# Autodesk Inventor assembly: Top PVC Roller
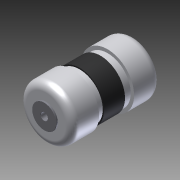
[picture p0: Inventor's stored thumbnail of the model, 180x180]
Saved by Autodesk Inventor 2014 SP1 (Build 180222100, 222)
## iProperties
Created: 2012-03-30
Part Number: Top PVC Roller
Document SubType Name: Assembly
Designer: Moses
Author: Moses
## Documents named in this file (5)
- C:\Users\Moses\Documents\Inventor\Rebuild\Repackaged_Team 3061_2012 Ball Shooter_Inventor Version_2014\Top PVC Roller.iam
- C:\Users\Moses\Documents\Inventor\Rebuild\Repackaged_Team 3061_2012 Ball Shooter_Inventor Version_2014\PVC Shooter Conveyor End Cap.ipt
- C:\Users\Moses\Documents\Inventor\Rebuild\Repackaged_Team 3061_2012 Ball Shooter_Inventor Version_2014\0.25 in Flanged Ball Bearing.ipt
- C:\Users\Moses\Documents\Inventor\Rebuild\Repackaged_Team 3061_2012 Ball Shooter_Inventor Version_2014\V5 Shooter Conveyor Roller.ipt
- C:\Users\Moses\Documents\Inventor\Rebuild\Repackaged_Team 3061_2012 Ball Shooter_Inventor Version_2014\PVC Rubber Covering.ipt
## Components (6 placed, 4 different names)
1. PVC Shooter Conveyor End Cap:1 — Insert:1, Mate:1, Mate:3, Mate:4, Mate:6
2. PVC Shooter Conveyor End Cap:2 — Insert:2, Mate:2, Mate:3
3. 0.25 in Flanged Ball Bearing:1 — Insert:1
4. 0.25 in Flanged Ball Bearing:2 — Insert:2
5. V5 Shooter Conveyor Roller:1 — Mate:1, Mate:2, Mate:4, Mate:5
6. PVC Rubber Covering:1 — Mate:5, Mate:6
## Relationships (8: Mate 6, Insert 2)
- Insert:1: PVC Shooter Conveyor End Cap:1 ↔ 0.25 in Flanged Ball Bearing:1
- Insert:2: PVC Shooter Conveyor End Cap:2 ↔ 0.25 in Flanged Ball Bearing:2
- Mate:1: PVC Shooter Conveyor End Cap:1 ↔ V5 Shooter Conveyor Roller:1
- Mate:2: PVC Shooter Conveyor End Cap:2 ↔ V5 Shooter Conveyor Roller:1
- Mate:3 (31.75 mm): PVC Shooter Conveyor End Cap:1 ↔ PVC Shooter Conveyor End Cap:2
- Mate:4 (1.905 mm): PVC Shooter Conveyor End Cap:1 ↔ V5 Shooter Conveyor Roller:1
- Mate:5: V5 Shooter Conveyor Roller:1 ↔ PVC Rubber Covering:1
- Mate:6 (6.35 mm): PVC Shooter Conveyor End Cap:1 ↔ PVC Rubber Covering:1
